# Autodesk Inventor assembly: NDV-2600 DrainSystemBottom 01
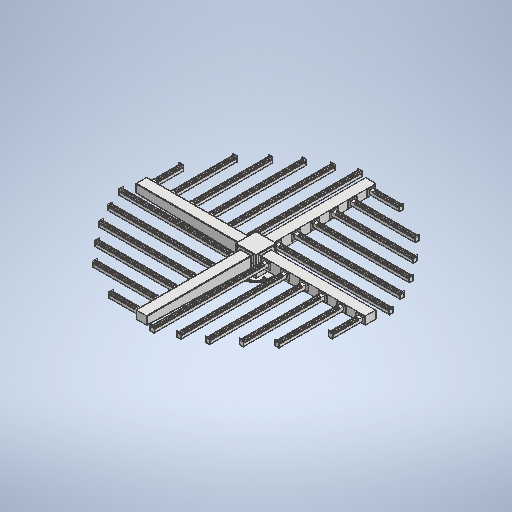
[picture p0: Inventor's stored thumbnail of the model, 512x512]
Saved by Autodesk Inventor 2026.2 (Build 302298000, 298)
## iProperties
Created: 2026-05-12
Part Number: NDV-2600 DrainSystemBottom 01
Document SubType Name: Assembly
Designer: admin
Stock Number: ДРС Ф2600
Mass: 111698 g
Surface Area: 133263 cm^2
Volume: 13962.3 cm^3
Density: 8 g/cm^3
Author: admin
## Documents named in this file (11)
- C:\Users\admin\Documents\Inventor\NDV-DistribSystem\DRS_D1200\NDV-2600 DrainSystemBottom 01.iam
- C:\Users\admin\Documents\Inventor\NDV-DistribSystem\DRS_D1200\NDV-0010 Parameters 01.ipt
- C:\Users\admin\Documents\Inventor\NDV-DistribSystem\DRS_D1200\NDV-1000 Center 01.iam
- C:\Users\admin\Documents\Inventor\NDV-DistribSystem\DRS_D1200\NDV-2000 Collector 01.iam
- C:\Users\admin\Documents\Inventor\NDV-DistribSystem\DRS_D1200\NDV-3100 Branch 1 01.iam
- C:\Users\admin\Documents\Inventor\NDV-DistribSystem\DRS_D1200\NDV-3200 Branch 2 01.iam
- C:\Users\admin\Documents\Inventor\NDV-DistribSystem\DRS_D1200\NDV-3300 Branch 3 01.iam
- C:\Users\admin\Documents\Inventor\NDV-DistribSystem\DRS_D1200\NDV-3400 Branch 4 01.iam
- C:\Users\admin\Documents\Inventor\NDV-DistribSystem\DRS_D1200\NDV-3500 Branch 5 01.iam
- C:\Users\admin\Documents\Inventor\NDV-DistribSystem\DRS_D1200\NDV-3600 Branch 6 01.iam
- C:\Users\admin\Documents\Inventor\NDV-DistribSystem\DRS_D1200\NDV-4000 Pipe flange 01.iam
## Components (32 placed, 10 different names)
1. NDV-0010 Parameters 01:1
2. NDV-0010 Parameters 01:2
3. NDV-1000 Center 01:1 [sub-assembly] — Mate:1, Mate:2, Mate:3, Mate:4, Mate:5, Mate:6, Mate:7, Mate:8, Mate:9, Mate:10, Mate:11, Mate:12, Mate:103, Flush:1, Mate:104
4. NDV-2000 Collector 01:1 [sub-assembly] — Mate:1, Mate:2, Mate:3, Mate:85, Mate:86, Mate:87, Mate:88, Mate:89, Mate:90, Mate:91, Mate:92, Mate:93, Mate:94, Mate:95, Mate:96, Mate:97, Mate:98, Mate:99, Mate:100, Mate:101, Mate:102
5. NDV-3100 Branch 1 01:1 [sub-assembly]
6. NDV-3200 Branch 2 01:1 [sub-assembly]
7. NDV-3300 Branch 3 01:1 [sub-assembly]
8. NDV-3400 Branch 4 01:1 [sub-assembly]
9. NDV-3500 Branch 5 01:1 [sub-assembly]
10. NDV-3600 Branch 6 01:1 [sub-assembly]
11. NDV-2000 Collector 01:2 [sub-assembly] — Mate:4, Mate:5, Mate:6
12. NDV-2000 Collector 01:3 [sub-assembly] — Mate:7, Mate:8, Mate:9, Mate:49, Mate:50, Mate:51, Mate:52, Mate:53, Mate:54, Mate:55, Mate:56, Mate:57, Mate:58, Mate:59, Mate:60, Mate:61, Mate:62, Mate:63, Mate:64, Mate:65, Mate:66
13. NDV-2000 Collector 01:4 [sub-assembly] — Mate:10, Mate:11, Mate:12, Mate:67, Mate:68, Mate:69, Mate:70, Mate:71, Mate:72, Mate:73, Mate:74, Mate:75, Mate:76, Mate:77, Mate:78, Mate:79, Mate:80, Mate:81, Mate:82, Mate:83, Mate:84
14. NDV-3100 Branch 1 01:3 [sub-assembly] — Mate:49, Mate:50, Mate:51
15. NDV-3200 Branch 2 01:3 [sub-assembly] — Mate:52, Mate:53, Mate:54
16. NDV-3300 Branch 3 01:3 [sub-assembly] — Mate:55, Mate:56, Mate:57
17. NDV-3400 Branch 4 01:3 [sub-assembly] — Mate:58, Mate:59, Mate:60
18. NDV-3500 Branch 5 01:3 [sub-assembly] — Mate:61, Mate:62, Mate:63
19. NDV-3600 Branch 6 01:3 [sub-assembly] — Mate:64, Mate:65, Mate:66
20. NDV-3100 Branch 1 01:4 [sub-assembly] — Mate:67, Mate:68, Mate:69
21. NDV-3200 Branch 2 01:4 [sub-assembly] — Mate:70, Mate:71, Mate:72
22. NDV-3300 Branch 3 01:4 [sub-assembly] — Mate:73, Mate:74, Mate:75
23. NDV-3400 Branch 4 01:4 [sub-assembly] — Mate:76, Mate:77, Mate:78
24. NDV-3500 Branch 5 01:4 [sub-assembly] — Mate:79, Mate:80, Mate:81
25. NDV-3600 Branch 6 01:4 [sub-assembly] — Mate:82, Mate:83, Mate:84
26. NDV-3100 Branch 1 01:5 [sub-assembly] — Mate:85, Mate:86, Mate:87
27. NDV-3200 Branch 2 01:5 [sub-assembly] — Mate:88, Mate:89, Mate:90
28. NDV-3300 Branch 3 01:5 [sub-assembly] — Mate:91, Mate:92, Mate:93
29. NDV-3400 Branch 4 01:5 [sub-assembly] — Mate:94, Mate:95, Mate:96
30. NDV-3500 Branch 5 01:5 [sub-assembly] — Mate:97, Mate:98, Mate:99
31. NDV-3600 Branch 6 01:5 [sub-assembly] — Mate:100, Mate:101, Mate:102
32. NDV-4000 Pipe flange 01:1 [sub-assembly] — Mate:103, Flush:1, Mate:104
## Relationships (87: Mate 86, Flush 1)
- Mate:1: NDV-1000 Center 01:1 ↔ NDV-2000 Collector 01:1
- Mate:2 (0.2 mm): NDV-1000 Center 01:1 ↔ NDV-2000 Collector 01:1
- Mate:3 (0.25 mm): NDV-1000 Center 01:1 ↔ NDV-2000 Collector 01:1
- Mate:4: NDV-1000 Center 01:1 ↔ NDV-2000 Collector 01:2
- Mate:5 (0.2 mm): NDV-1000 Center 01:1 ↔ NDV-2000 Collector 01:2
- Mate:6 (0.25 mm): NDV-1000 Center 01:1 ↔ NDV-2000 Collector 01:2
- Mate:7: NDV-1000 Center 01:1 ↔ NDV-2000 Collector 01:3
- Mate:8 (0.2 mm): NDV-1000 Center 01:1 ↔ NDV-2000 Collector 01:3
- Mate:9 (0.3 mm): NDV-1000 Center 01:1 ↔ NDV-2000 Collector 01:3
- Mate:10: NDV-1000 Center 01:1 ↔ NDV-2000 Collector 01:4
- Mate:11 (0.3 mm): NDV-1000 Center 01:1 ↔ NDV-2000 Collector 01:4
- Mate:12 (0.3 mm): NDV-1000 Center 01:1 ↔ NDV-2000 Collector 01:4
- [Mate]: NDV-3100 Branch 1 01:1 ↔ NDV-2000 Collector 01:2
- [Mate] (0.25 mm): NDV-3100 Branch 1 01:1 ↔ NDV-2000 Collector 01:2
- [Mate] (0.25 mm): NDV-3100 Branch 1 01:1 ↔ NDV-2000 Collector 01:2
- [Mate]: NDV-3200 Branch 2 01:1 ↔ NDV-2000 Collector 01:2
- [Mate] (0.25 mm): NDV-3200 Branch 2 01:1 ↔ NDV-2000 Collector 01:2
- [Mate] (0.25 mm): NDV-3200 Branch 2 01:1 ↔ NDV-2000 Collector 01:2
- [Mate]: NDV-3300 Branch 3 01:1 ↔ NDV-2000 Collector 01:2
- [Mate] (0.25 mm): NDV-3300 Branch 3 01:1 ↔ NDV-2000 Collector 01:2
- [Mate] (0.25 mm): NDV-3300 Branch 3 01:1 ↔ NDV-2000 Collector 01:2
- [Mate]: NDV-3400 Branch 4 01:1 ↔ NDV-2000 Collector 01:2
- [Mate] (0.25 mm): NDV-3400 Branch 4 01:1 ↔ NDV-2000 Collector 01:2
- [Mate] (0.25 mm): NDV-3400 Branch 4 01:1 ↔ NDV-2000 Collector 01:2
- [Mate]: NDV-3500 Branch 5 01:1 ↔ NDV-2000 Collector 01:2
- [Mate] (0.25 mm): NDV-3500 Branch 5 01:1 ↔ NDV-2000 Collector 01:2
- [Mate] (0.25 mm): NDV-3500 Branch 5 01:1 ↔ NDV-2000 Collector 01:2
- [Mate]: NDV-3600 Branch 6 01:1 ↔ NDV-2000 Collector 01:2
- [Mate] (0.25 mm): NDV-3600 Branch 6 01:1 ↔ NDV-2000 Collector 01:2
- [Mate] (0.25 mm): NDV-3600 Branch 6 01:1 ↔ NDV-2000 Collector 01:2
- Mate:49: NDV-2000 Collector 01:3 ↔ NDV-3100 Branch 1 01:3
- Mate:50 (0.25 mm): NDV-2000 Collector 01:3 ↔ NDV-3100 Branch 1 01:3
- Mate:51 (0.25 mm): NDV-2000 Collector 01:3 ↔ NDV-3100 Branch 1 01:3
- Mate:52: NDV-2000 Collector 01:3 ↔ NDV-3200 Branch 2 01:3
- Mate:53 (0.25 mm): NDV-2000 Collector 01:3 ↔ NDV-3200 Branch 2 01:3
- Mate:54 (0.25 mm): NDV-2000 Collector 01:3 ↔ NDV-3200 Branch 2 01:3
- Mate:55: NDV-2000 Collector 01:3 ↔ NDV-3300 Branch 3 01:3
- Mate:56 (0.25 mm): NDV-2000 Collector 01:3 ↔ NDV-3300 Branch 3 01:3
- Mate:57 (0.25 mm): NDV-2000 Collector 01:3 ↔ NDV-3300 Branch 3 01:3
- Mate:58: NDV-2000 Collector 01:3 ↔ NDV-3400 Branch 4 01:3
- Mate:59 (0.25 mm): NDV-2000 Collector 01:3 ↔ NDV-3400 Branch 4 01:3
- Mate:60 (0.25 mm): NDV-2000 Collector 01:3 ↔ NDV-3400 Branch 4 01:3
- Mate:61: NDV-2000 Collector 01:3 ↔ NDV-3500 Branch 5 01:3
- Mate:62 (0.25 mm): NDV-2000 Collector 01:3 ↔ NDV-3500 Branch 5 01:3
- Mate:63 (0.25 mm): NDV-2000 Collector 01:3 ↔ NDV-3500 Branch 5 01:3
- Mate:64: NDV-2000 Collector 01:3 ↔ NDV-3600 Branch 6 01:3
- Mate:65 (0.25 mm): NDV-2000 Collector 01:3 ↔ NDV-3600 Branch 6 01:3
- Mate:66 (0.25 mm): NDV-2000 Collector 01:3 ↔ NDV-3600 Branch 6 01:3
- Mate:67: NDV-2000 Collector 01:4 ↔ NDV-3100 Branch 1 01:4
- Mate:68 (0.25 mm): NDV-2000 Collector 01:4 ↔ NDV-3100 Branch 1 01:4
- Mate:69 (0.25 mm): NDV-2000 Collector 01:4 ↔ NDV-3100 Branch 1 01:4
- Mate:70: NDV-2000 Collector 01:4 ↔ NDV-3200 Branch 2 01:4
- Mate:71 (0.25 mm): NDV-2000 Collector 01:4 ↔ NDV-3200 Branch 2 01:4
- Mate:72 (0.25 mm): NDV-2000 Collector 01:4 ↔ NDV-3200 Branch 2 01:4
- Mate:73: NDV-2000 Collector 01:4 ↔ NDV-3300 Branch 3 01:4
- Mate:74 (0.25 mm): NDV-2000 Collector 01:4 ↔ NDV-3300 Branch 3 01:4
- Mate:75 (0.25 mm): NDV-2000 Collector 01:4 ↔ NDV-3300 Branch 3 01:4
- Mate:76: NDV-2000 Collector 01:4 ↔ NDV-3400 Branch 4 01:4
- Mate:77 (0.25 mm): NDV-2000 Collector 01:4 ↔ NDV-3400 Branch 4 01:4
- Mate:78 (0.25 mm): NDV-2000 Collector 01:4 ↔ NDV-3400 Branch 4 01:4
- Mate:79: NDV-2000 Collector 01:4 ↔ NDV-3500 Branch 5 01:4
- Mate:80 (0.25 mm): NDV-2000 Collector 01:4 ↔ NDV-3500 Branch 5 01:4
- Mate:81 (0.25 mm): NDV-2000 Collector 01:4 ↔ NDV-3500 Branch 5 01:4
- Mate:82: NDV-2000 Collector 01:4 ↔ NDV-3600 Branch 6 01:4
- Mate:83 (0.25 mm): NDV-2000 Collector 01:4 ↔ NDV-3600 Branch 6 01:4
- Mate:84 (0.25 mm): NDV-2000 Collector 01:4 ↔ NDV-3600 Branch 6 01:4
- Mate:85: NDV-2000 Collector 01:1 ↔ NDV-3100 Branch 1 01:5
- Mate:86 (0.25 mm): NDV-2000 Collector 01:1 ↔ NDV-3100 Branch 1 01:5
- Mate:87 (0.25 mm): NDV-2000 Collector 01:1 ↔ NDV-3100 Branch 1 01:5
- Mate:88: NDV-2000 Collector 01:1 ↔ NDV-3200 Branch 2 01:5
- Mate:89 (0.25 mm): NDV-2000 Collector 01:1 ↔ NDV-3200 Branch 2 01:5
- Mate:90 (0.25 mm): NDV-2000 Collector 01:1 ↔ NDV-3200 Branch 2 01:5
- Mate:91: NDV-2000 Collector 01:1 ↔ NDV-3300 Branch 3 01:5
- Mate:92 (0.25 mm): NDV-2000 Collector 01:1 ↔ NDV-3300 Branch 3 01:5
- Mate:93 (0.25 mm): NDV-2000 Collector 01:1 ↔ NDV-3300 Branch 3 01:5
- Mate:94: NDV-2000 Collector 01:1 ↔ NDV-3400 Branch 4 01:5
- Mate:95 (0.25 mm): NDV-2000 Collector 01:1 ↔ NDV-3400 Branch 4 01:5
- Mate:96 (0.25 mm): NDV-2000 Collector 01:1 ↔ NDV-3400 Branch 4 01:5
- Mate:97: NDV-2000 Collector 01:1 ↔ NDV-3500 Branch 5 01:5
- Mate:98 (0.25 mm): NDV-2000 Collector 01:1 ↔ NDV-3500 Branch 5 01:5
- Mate:99 (0.25 mm): NDV-2000 Collector 01:1 ↔ NDV-3500 Branch 5 01:5
- Mate:100: NDV-2000 Collector 01:1 ↔ NDV-3600 Branch 6 01:5
- Mate:101 (0.25 mm): NDV-2000 Collector 01:1 ↔ NDV-3600 Branch 6 01:5
- Mate:102 (0.25 mm): NDV-2000 Collector 01:1 ↔ NDV-3600 Branch 6 01:5
- Mate:103: NDV-1000 Center 01:1 ↔ NDV-4000 Pipe flange 01:1
- Flush:1: NDV-1000 Center 01:1 ↔ NDV-4000 Pipe flange 01:1
- Mate:104: NDV-1000 Center 01:1 ↔ NDV-4000 Pipe flange 01:1
